# Autodesk Inventor assembly: wildfire
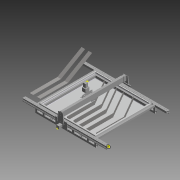
[picture p0: Inventor's stored thumbnail of the model, 180x180]
Saved by Autodesk Inventor 2013 (Build 170138000, 138)
## iProperties
Created: 2012-11-30
Part Number: wildfire
Document SubType Name: Assembly
Designer: istvan.burbank
Mass: 35060.2 g
Surface Area: 149069 cm^2
Volume: 21794.8 cm^3
Density: 1.60865 g/cm^3
Author: istvan.burbank
## Documents named in this file (6)
- D:\GitHub\Crown-Fire\CAD\wildfire.iam
- D:\GitHub\Crown-Fire\CAD\Frame\frame.iam
- D:\GitHub\Crown-Fire\CAD\GantryMount\tractor.iam
- D:\GitHub\Crown-Fire\CAD\Gantry\gantry.iam
- D:\GitHub\Crown-Fire\CAD\Carriage\carriage.iam
- D:\GitHub\Crown-Fire\CAD\CuttingHead\CuttingHead.iam
## Components (6 placed, 5 different names)
1. frame:1 [sub-assembly] — Tangent:1, Tangent:2, Tangent:3, Tangent:4, Tangent:5, Tangent:6
2. tractor:1 [sub-assembly] — Tangent:1, Tangent:2, Tangent:3, Mate:8, Mate:9
3. tractor:2 [sub-assembly] — Tangent:4, Tangent:5, Tangent:6, Mate:4, Mate:6, Mate:7
4. gantry:1 [sub-assembly] — Mate:4, Tangent:7, Tangent:8, Tangent:9, Mate:6, Mate:7, Mate:8, Mate:9
5. carriage:1 [sub-assembly] — Tangent:7, Tangent:8, Tangent:9, Mate:10, Angle:1
6. CuttingHead:1 [sub-assembly] — Mate:10, Angle:1
## Relationships (16: Tangent 9, Mate 6, Angle 1)
- Tangent:1: frame:1 ↔ tractor:1
- Tangent:2: frame:1 ↔ tractor:1
- Tangent:3: frame:1 ↔ tractor:1
- Tangent:4: frame:1 ↔ tractor:2
- Tangent:5: frame:1 ↔ tractor:2
- Tangent:6: frame:1 ↔ tractor:2
- Mate:4: tractor:2 ↔ gantry:1
- Tangent:7: gantry:1 ↔ carriage:1
- Tangent:8: gantry:1 ↔ carriage:1
- Tangent:9: gantry:1 ↔ carriage:1
- Mate:6: tractor:2 ↔ gantry:1
- Mate:7: tractor:2 ↔ gantry:1
- Mate:8: tractor:1 ↔ gantry:1
- Mate:9: tractor:1 ↔ gantry:1
- Mate:10: carriage:1 ↔ CuttingHead:1
- Angle:1 (0 deg): carriage:1 ↔ CuttingHead:1
